# Autodesk Inventor assembly: New Box ARm
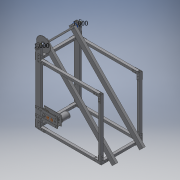
[picture p0: Inventor's stored thumbnail of the model, 180x180]
Saved by Autodesk Inventor 2018 (Build 220112000, 112)
## iProperties
Created: 2019-01-24
Part Number: New Box ARm
Document SubType Name: Assembly
Designer: Gabriel
Author: Gabriel
## Documents named in this file (18)
- C:\Users\Gabriel\Documents\GitHub\2019CAD\New ARm Box\New Box ARm.iam
- C:\Users\Gabriel\Documents\GitHub\2019CAD\New ARm Box\30in Vertical 1x2 Beam.ipt
- C:\Users\Gabriel\Documents\GitHub\2019CAD\New ARm Box\24in Vertical 1x1 Beam.ipt
- C:\Users\Gabriel\Documents\GitHub\2019CAD\New ARm Box\15in Horizontal 1x1 Beam.ipt
- C:\Users\Gabriel\Documents\GitHub\2019CAD\New ARm Box\24in Horizontal 1x1 Beam.ipt
- C:\Users\Gabriel\Documents\GitHub\2019CAD\New ARm Box\25in Horizontal 1x1 Beam.ipt
- C:\Users\Gabriel\Documents\GitHub\2019CAD\New ARm Box\ARm Gearbox.iam
- C:\Users\Gabriel\Documents\GitHub\2019CAD\New ARm Box\L gusset.ipt
- C:\Users\Gabriel\Documents\GitHub\2019CAD\New ARm Box\1_2_Acetal_Spacer_-_1_2_Hex_217-3261.ipt
- C:\Users\Gabriel\Documents\GitHub\2019CAD\New ARm Box\Clamping_Shaft_Collar_-_1_2_Hex_ID_217-2737.ipt
- C:\Users\Gabriel\Documents\GitHub\2019CAD\New ARm Box\_72t_Aluminum_Plate_Sprocket_25_Chain_1-1_8_Bearing_Bore_217-2627.ipt
- C:\Users\Gabriel\Documents\GitHub\2019CAD\New ARm Box\0_500_ID_x_1_125_OD_x_0_313_WD_Flanged_Bearing_217-2731.ipt
- C:\Users\Gabriel\Documents\GitHub\2019CAD\New ARm Box\41.75in Arm Beam.ipt
- C:\Users\Gabriel\Documents\GitHub\2019CAD\New ARm Box\Hex Hub.ipt
- C:\Users\Gabriel\Documents\GitHub\2019CAD\New ARm Box\Hex Shaft ARm.ipt
- C:\Users\Gabriel\Documents\GitHub\2019CAD\New ARm Box\.75in 92196A245_18-8 STAINLESS STEEL SOCKET HEAD CAP SCREW.ipt
- C:\Users\Gabriel\Documents\GitHub\2019CAD\New ARm Box\1.5in 92196A251_18-8 STAINLESS STEEL SOCKET HEAD CAP SCREW.ipt
- C:\Users\Gabriel\Downloads\LV Gusset.ipt
## Components (105 placed, 17 different names)
1. 30in Vertical 1x2 Beam:1 — Mate:4, Mate:5, Mate:6, Flush:6, Flush:17, Mate:27, Mate:30, Flush:19, Flush:21, Flush:31, Mate:38, Mate:39, Flush:35, Mate:41, Flush:43, Flush:44, Mate:53, Mate:54, Mate:55, Mate:56, Mate:57, Flush:60, Mate:58, Mate:60, Mate:61, Mate:62, Flush:61, Mate:65, Mate:67, Mate:68, Mate:69, Flush:64, Mate:79, Mate:81, Mate:82, Mate:83, Flush:68, Mate:93, Mate:95, Mate:96, Mate:97, Flush:72, Mate:168, Mate:177, Mate:178, Mate:179, Flush:110, Flush:114, Flush:118, Mate:184, Mate:186, Mate:187, Mate:188, Flush:122, Flush:125, Mate:196, Mate:197, Mate:198, Mate:199
2. 30in Vertical 1x2 Beam:2 — Mate:7, Mate:8, Mate:9, Flush:5, Flush:18, Mate:33, Mate:35, Flush:25, Flush:27, Flush:31, Mate:37, Mate:40, Flush:34, Mate:47, Flush:49, Flush:50, Mate:72, Mate:74, Mate:75, Mate:76, Flush:66, Mate:86, Mate:88, Mate:89, Mate:90, Flush:70, Mate:100, Mate:102, Mate:103, Mate:104, Flush:74, Mate:107, Mate:109, Mate:110, Mate:111, Flush:76, Mate:170, Mate:172, Mate:173, Mate:174, Flush:112, Flush:116, Flush:117, Mate:182, Mate:191, Mate:192, Mate:193, Flush:120, Flush:126, Mate:200, Mate:201, Mate:202, Mate:203
3. 24in Vertical 1x1 Beam:3 — Flush:13, Flush:16, Flush:17, Mate:28, Mate:29, Flush:20, Flush:22, Flush:23, Mate:31, Flush:39, Mate:45, Mate:46, Flush:40, Mate:114, Flush:78, Flush:79, Mate:128, Flush:84, Flush:85, Mate:156, Mate:158, Mate:159, Flush:100, Flush:103, Mate:300, Mate:304, Mate:305, Flush:134, Flush:135
4. 24in Vertical 1x1 Beam:4 — Flush:16, Flush:18, Mate:32, Mate:34, Flush:24, Flush:26, Flush:32, Mate:36, Mate:51, Mate:52, Flush:46, Flush:47, Mate:121, Flush:81, Flush:82, Mate:135, Flush:87, Flush:88, Mate:162, Mate:164, Mate:165, Flush:105, Flush:108, Mate:306, Mate:310, Mate:311, Flush:130, Flush:131
5. 15in Horizontal 1x1 Beam:1 — Flush:13, Flush:30, Mate:42, Mate:43, Mate:44, Flush:41, Flush:42, Mate:48, Flush:45, Mate:49, Mate:50, Flush:48, Flush:52, Flush:53, Flush:56, Mate:157, Mate:160, Mate:161, Flush:99, Flush:101, Mate:163, Mate:166, Mate:167, Flush:104, Flush:106, Mate:242
6. 15in Horizontal 1x1 Beam:2 — Mate:4, Mate:5, Mate:6, Mate:7, Mate:8, Mate:9, Flush:5, Flush:6, Flush:30, Flush:38, Flush:54, Flush:55, Flush:56, Mate:169, Mate:171, Mate:175, Mate:176, Mate:180, Mate:181, Flush:109, Flush:111, Flush:113, Flush:115
7. 15in Horizontal 1x1 Beam:3 — Mate:37, Mate:38, Mate:39, Mate:40, Flush:34, Flush:35, Flush:36, Flush:37, Flush:38, Mate:183, Mate:185, Mate:189, Mate:190, Mate:194, Mate:195, Flush:119, Flush:121, Flush:123, Flush:124
8. 24in Horizontal 1x1 Beam:1 — Mate:32, Mate:33, Mate:34, Mate:35, Flush:24, Flush:25, Flush:26, Flush:27, Flush:32, Mate:36, Flush:33, Flush:37, Flush:58, Mate:73, Mate:77, Mate:78, Flush:65, Mate:87, Mate:91, Mate:92, Flush:69, Mate:122, Mate:123, Mate:124, Flush:80, Mate:136, Mate:137, Mate:138, Flush:86
9. 24in Horizontal 1x1 Beam:2 — Mate:27, Mate:28, Mate:29, Mate:30, Flush:19, Flush:20, Flush:21, Flush:22, Flush:23, Mate:31, Flush:33, Flush:36, Flush:57, Mate:66, Mate:70, Mate:71, Flush:63, Mate:80, Mate:84, Mate:85, Flush:67, Mate:115, Mate:116, Mate:117, Flush:77, Mate:129, Mate:130, Mate:131, Flush:83
10. 25in Horizontal 1x1 Beam:1 — Mate:41, Flush:39, Mate:42, Mate:43, Mate:44, Mate:45, Mate:46, Flush:40, Flush:41, Flush:42, Flush:43, Flush:44, Flush:51, Flush:53, Flush:55, Flush:57, Flush:59, Mate:59, Flush:62, Mate:94, Flush:71, Flush:102, Mate:301, Mate:302, Mate:303, Flush:133, Flush:136
11. 25in Horizontal 1x1 Beam:2 — Mate:47, Mate:48, Flush:45, Mate:49, Mate:50, Mate:51, Mate:52, Flush:46, Flush:47, Flush:48, Flush:49, Flush:50, Flush:51, Flush:52, Flush:54, Flush:58, Flush:59, Mate:101, Flush:73, Mate:108, Flush:75, Flush:107, Mate:307, Mate:308, Mate:309, Flush:129, Flush:132
12. ARm Gearbox:1 [sub-assembly] — Mate:53, Mate:54, Mate:55, Mate:56, Mate:57, Flush:60
13. L gusset:1 — Mate:93, Mate:94, Mate:95, Mate:96, Mate:97, Flush:71, Flush:72
14. L gusset:2 — Mate:100, Mate:101, Mate:102, Mate:103, Mate:104, Flush:73, Flush:74
15. L gusset:5 — Mate:114, Mate:115, Mate:116, Mate:117, Flush:77, Flush:78, Flush:79
16. L gusset:6 — Mate:121, Mate:122, Mate:123, Mate:124, Flush:80, Flush:81, Flush:82
17. L gusset:7 — Mate:72, Mate:73, Mate:74, Mate:75, Mate:76, Mate:77, Mate:78, Flush:65, Flush:66
18. L gusset:8 — Mate:65, Mate:66, Mate:67, Mate:68, Mate:69, Mate:70, Mate:71, Flush:63, Flush:64, Mate:273, Mate:274, Mate:275, Mate:277, Mate:289, Mate:291, Mate:292, Mate:293, Mate:382, Mate:383
19. L gusset:9 — Mate:58, Mate:59, Mate:60, Mate:61, Mate:62, Flush:61, Flush:62, Mate:259, Mate:260, Mate:261, Mate:263, Mate:285, Mate:286, Mate:287, Mate:288
20. L gusset:10 — Mate:107, Mate:108, Mate:109, Mate:110, Mate:111, Flush:75, Flush:76, Mate:296, Mate:297, Mate:298, Mate:328, Mate:329, Mate:330, Mate:337, Mate:338
21. L gusset:11 — Mate:86, Mate:87, Mate:88, Mate:89, Mate:90, Mate:91, Mate:92, Flush:69, Flush:70, Mate:364, Mate:365, Mate:366, Mate:368, Mate:369, Mate:370, Mate:372, Mate:373, Mate:380, Mate:381
22. L gusset:12 — Mate:79, Mate:80, Mate:81, Mate:82, Mate:83, Mate:84, Mate:85, Flush:67, Flush:68
23. L gusset:13 — Mate:135, Mate:136, Mate:137, Mate:138, Flush:86, Flush:87, Flush:88, Mate:332, Mate:333, Mate:334, Mate:335, Mate:336, Mate:359, Mate:360, Mate:361, Mate:362, Mate:363
24. L gusset:14 — Mate:128, Mate:129, Mate:130, Mate:131, Flush:83, Flush:84, Flush:85, Mate:268, Mate:269, Mate:270, Mate:271, Mate:272, Mate:278, Mate:279, Mate:280, Mate:281, Mate:282
25. L gusset:15 — Mate:168, Mate:169, Mate:177, Mate:178, Mate:179, Mate:180, Mate:181, Flush:109, Flush:110, Flush:113, Flush:114, Flush:118, Mate:339, Mate:340, Mate:341, Mate:342, Mate:349, Mate:350
26. L gusset:16 — Mate:156, Mate:157, Mate:158, Mate:159, Mate:160, Mate:161, Flush:99, Flush:100, Flush:101, Flush:102, Flush:103, Mate:351, Mate:352, Mate:357, Mate:358
27. L gusset:17 — Mate:184, Mate:185, Mate:186, Mate:187, Mate:188, Mate:189, Mate:190, Flush:121, Flush:122, Flush:123, Flush:125, Mate:376, Mate:377, Mate:388, Mate:389, Mate:390, Mate:391, Mate:394, Mate:395, Mate:400, Mate:401
28. L gusset:18 — Mate:162, Mate:163, Mate:164, Mate:165, Mate:166, Mate:167, Flush:104, Flush:105, Flush:106, Flush:107, Flush:108, Mate:353, Mate:354, Mate:355, Mate:356
29. L gusset:19 — Mate:170, Mate:171, Mate:172, Mate:173, Mate:174, Mate:175, Mate:176, Flush:111, Flush:112, Flush:115, Flush:116, Flush:117, Mate:343, Mate:344, Mate:345, Mate:346, Mate:347, Mate:348
30. L gusset:20 — Mate:182, Mate:183, Mate:191, Mate:192, Mate:193, Mate:194, Mate:195, Flush:119, Flush:120, Flush:124, Flush:126, Mate:384, Mate:385, Mate:386, Mate:387, Mate:392, Mate:393, Mate:396, Mate:397, Mate:398, Mate:399
31. 1_2_Acetal_Spacer_-_1_2_Hex_217-3261:1 — Mate:213, Mate:214, Mate:215, Mate:216
32. Clamping_Shaft_Collar_-_1_2_Hex_ID_217-2737:1 — Mate:204, Mate:205, Flush:127, Mate:208
33. _72t_Aluminum_Plate_Sprocket_25_Chain_1-1_8_Bearing_Bore_217-2627:1 — Mate:217, Mate:218, Mate:219, Mate:220, Mate:221
34. 0_500_ID_x_1_125_OD_x_0_313_WD_Flanged_Bearing_217-2731:1 — Mate:196, Mate:197, Mate:209, Mate:210
35. 1_2_Acetal_Spacer_-_1_2_Hex_217-3261:2 — Mate:206, Mate:207, Mate:208, Mate:209, Mate:210
36. 41.75in Arm Beam:1 — Mate:222, Mate:229, Flush:128, Rotation:3, Mate:242
37. 0_500_ID_x_1_125_OD_x_0_313_WD_Flanged_Bearing_217-2731:2 — Mate:198, Mate:199, Mate:215
38. Hex Hub:1 — Mate:211, Mate:212, Mate:216, Mate:217, Mate:218, Mate:219, Mate:220, Mate:221, Mate:226
39. Hex Hub:2 — Mate:222, Mate:224, Mate:225, Mate:226, Mate:229, Rotation:3, Rotation:4
40. Hex Shaft ARm:1 — Mate:204, Mate:205, Flush:127, Mate:206, Mate:207, Mate:211, Mate:212, Mate:213, Mate:214, Mate:224, Mate:225, Mate:230, Mate:231, Mate:233, Mate:234, Mate:236, Mate:237, Mate:240, Mate:241, Rotation:2, Rotation:4
41. 41.75in Arm Beam:2 — Mate:227, Mate:228, Rotation:1, Flush:128
42. Hex Hub:3 — Mate:227, Mate:228, Mate:239, Mate:240, Mate:241, Rotation:1, Rotation:2
43. 1_2_Acetal_Spacer_-_1_2_Hex_217-3261:4 — Mate:230, Mate:231, Mate:232, Mate:239
44. 0_500_ID_x_1_125_OD_x_0_313_WD_Flanged_Bearing_217-2731:3 — Mate:201, Mate:203, Mate:232
45. 0_500_ID_x_1_125_OD_x_0_313_WD_Flanged_Bearing_217-2731:4 — Mate:200, Mate:202, Mate:235
46. 1_2_Acetal_Spacer_-_1_2_Hex_217-3261:6 — Mate:233, Mate:234, Mate:235, Mate:238
47. Clamping_Shaft_Collar_-_1_2_Hex_ID_217-2737:2 — Mate:236, Mate:237, Mate:238
48. .75in 92196A245_18-8 STAINLESS STEEL SOCKET HEAD CAP SCREW:1 — Mate:376, Mate:377
49. 1.5in 92196A251_18-8 STAINLESS STEEL SOCKET HEAD CAP SCREW:1 — Mate:320, Mate:322
50. 1.5in 92196A251_18-8 STAINLESS STEEL SOCKET HEAD CAP SCREW:2 — Mate:317, Mate:319
51. 1.5in 92196A251_18-8 STAINLESS STEEL SOCKET HEAD CAP SCREW:3 — Mate:324, Mate:327
52. 1.5in 92196A251_18-8 STAINLESS STEEL SOCKET HEAD CAP SCREW:5 — Mate:341, Mate:350
53. 1.5in 92196A251_18-8 STAINLESS STEEL SOCKET HEAD CAP SCREW:6 — Mate:364, Mate:369
54. 1.5in 92196A251_18-8 STAINLESS STEEL SOCKET HEAD CAP SCREW:7 — Mate:312, Mate:315
55. 1.5in 92196A251_18-8 STAINLESS STEEL SOCKET HEAD CAP SCREW:8 — Mate:325, Mate:326
56. 1.5in 92196A251_18-8 STAINLESS STEEL SOCKET HEAD CAP SCREW:9 — Mate:271, Mate:281
57. 1.5in 92196A251_18-8 STAINLESS STEEL SOCKET HEAD CAP SCREW:10 — Mate:270, Mate:280
58. 1.5in 92196A251_18-8 STAINLESS STEEL SOCKET HEAD CAP SCREW:11 — Mate:313, Mate:314
59. 1.5in 92196A251_18-8 STAINLESS STEEL SOCKET HEAD CAP SCREW:12 — Mate:332, Mate:361
60. 1.5in 92196A251_18-8 STAINLESS STEEL SOCKET HEAD CAP SCREW:13 — Mate:259, Mate:288
61. .75in 92196A245_18-8 STAINLESS STEEL SOCKET HEAD CAP SCREW:14 — Mate:386, Mate:392
62. 1.5in 92196A251_18-8 STAINLESS STEEL SOCKET HEAD CAP SCREW:14 — Mate:316, Mate:318
63. .75in 92196A245_18-8 STAINLESS STEEL SOCKET HEAD CAP SCREW:15 — Mate:387, Mate:393
64. 1.5in 92196A251_18-8 STAINLESS STEEL SOCKET HEAD CAP SCREW:15 — Mate:297, Mate:329
65. .75in 92196A245_18-8 STAINLESS STEEL SOCKET HEAD CAP SCREW:17 — Mate:388, Mate:390
66. 1.5in 92196A251_18-8 STAINLESS STEEL SOCKET HEAD CAP SCREW:17 — Mate:298, Mate:330
67. 1.5in 92196A251_18-8 STAINLESS STEEL SOCKET HEAD CAP SCREW:18 — Mate:336, Mate:363
68. 1.5in 92196A251_18-8 STAINLESS STEEL SOCKET HEAD CAP SCREW:19 — Mate:366, Mate:372
69. 1.5in 92196A251_18-8 STAINLESS STEEL SOCKET HEAD CAP SCREW:20 — Mate:321, Mate:323
70. 1.5in 92196A251_18-8 STAINLESS STEEL SOCKET HEAD CAP SCREW:21 — Mate:339, Mate:340
71. 1.5in 92196A251_18-8 STAINLESS STEEL SOCKET HEAD CAP SCREW:22 — Mate:334, Mate:359
72. 1.5in 92196A251_18-8 STAINLESS STEEL SOCKET HEAD CAP SCREW:24 — Mate:261, Mate:286
73. 1.5in 92196A251_18-8 STAINLESS STEEL SOCKET HEAD CAP SCREW:25 — Mate:275, Mate:291
74. 1.5in 92196A251_18-8 STAINLESS STEEL SOCKET HEAD CAP SCREW:26 — Mate:333, Mate:360
75. 1.5in 92196A251_18-8 STAINLESS STEEL SOCKET HEAD CAP SCREW:27 — Mate:365, Mate:370
76. 1.5in 92196A251_18-8 STAINLESS STEEL SOCKET HEAD CAP SCREW:28 — Mate:337, Mate:338
77. 1.5in 92196A251_18-8 STAINLESS STEEL SOCKET HEAD CAP SCREW:30 — Mate:335, Mate:362
78. 1.5in 92196A251_18-8 STAINLESS STEEL SOCKET HEAD CAP SCREW:31 — Mate:368, Mate:373
79. 1.5in 92196A251_18-8 STAINLESS STEEL SOCKET HEAD CAP SCREW:33 — Mate:395, Mate:401
80. .75in 92196A245_18-8 STAINLESS STEEL SOCKET HEAD CAP SCREW:34 — Mate:384, Mate:385
81. 1.5in 92196A251_18-8 STAINLESS STEEL SOCKET HEAD CAP SCREW:34 — Mate:296, Mate:328
82. 1.5in 92196A251_18-8 STAINLESS STEEL SOCKET HEAD CAP SCREW:35 — Mate:273, Mate:293
83. 1.5in 92196A251_18-8 STAINLESS STEEL SOCKET HEAD CAP SCREW:36 — Mate:274, Mate:292
84. 1.5in 92196A251_18-8 STAINLESS STEEL SOCKET HEAD CAP SCREW:38 — Mate:263, Mate:287
85. 1.5in 92196A251_18-8 STAINLESS STEEL SOCKET HEAD CAP SCREW:39 — Mate:260, Mate:285
86. 1.5in 92196A251_18-8 STAINLESS STEEL SOCKET HEAD CAP SCREW:43 — Mate:277, Mate:289
87. 1.5in 92196A251_18-8 STAINLESS STEEL SOCKET HEAD CAP SCREW:45 — Mate:272, Mate:282
88. 1.5in 92196A251_18-8 STAINLESS STEEL SOCKET HEAD CAP SCREW:47 — Mate:269, Mate:278
89. 1.5in 92196A251_18-8 STAINLESS STEEL SOCKET HEAD CAP SCREW:49 — Mate:268, Mate:279
90. 1.5in 92196A251_18-8 STAINLESS STEEL SOCKET HEAD CAP SCREW:50 — Mate:397, Mate:399
91. 1.5in 92196A251_18-8 STAINLESS STEEL SOCKET HEAD CAP SCREW:51 — Mate:343, Mate:348
92. 1.5in 92196A251_18-8 STAINLESS STEEL SOCKET HEAD CAP SCREW:52 — Mate:342, Mate:349
93. 1.5in 92196A251_18-8 STAINLESS STEEL SOCKET HEAD CAP SCREW:54 — Mate:394, Mate:400
94. 1.5in 92196A251_18-8 STAINLESS STEEL SOCKET HEAD CAP SCREW:56 — Mate:396, Mate:398
95. LV Gusset:1 — Mate:306, Mate:307, Mate:308, Mate:309, Mate:310, Mate:311, Flush:129, Flush:130, Flush:131, Flush:132, Mate:320, Mate:321, Mate:322, Mate:323, Mate:324, Mate:325, Mate:326, Mate:327
96. LV Gusset:2 — Mate:300, Mate:301, Mate:302, Mate:303, Mate:304, Mate:305, Flush:133, Flush:134, Flush:135, Flush:136, Mate:312, Mate:313, Mate:314, Mate:315, Mate:316, Mate:317, Mate:318, Mate:319
97. 1.5in 92196A251_18-8 STAINLESS STEEL SOCKET HEAD CAP SCREW:58 — Mate:344, Mate:347
98. 1.5in 92196A251_18-8 STAINLESS STEEL SOCKET HEAD CAP SCREW:59 — Mate:345, Mate:346
99. 1.5in 92196A251_18-8 STAINLESS STEEL SOCKET HEAD CAP SCREW:60 — Mate:354, Mate:355
100. 1.5in 92196A251_18-8 STAINLESS STEEL SOCKET HEAD CAP SCREW:61 — Mate:352, Mate:358
101. 1.5in 92196A251_18-8 STAINLESS STEEL SOCKET HEAD CAP SCREW:64 — Mate:353, Mate:356
102. 1.5in 92196A251_18-8 STAINLESS STEEL SOCKET HEAD CAP SCREW:67 — Mate:351, Mate:357
103. 1.5in 92196A251_18-8 STAINLESS STEEL SOCKET HEAD CAP SCREW:68 — Mate:380, Mate:381
104. 1.5in 92196A251_18-8 STAINLESS STEEL SOCKET HEAD CAP SCREW:69 — Mate:382, Mate:383
105. .75in 92196A245_18-8 STAINLESS STEEL SOCKET HEAD CAP SCREW:58 — Mate:389, Mate:391
## Relationships (427: Mate 311, Flush 112, RelateRotation 4)
- Mate:4: 30in Vertical 1x2 Beam:1 ↔ 15in Horizontal 1x1 Beam:2
- Mate:5: 30in Vertical 1x2 Beam:1 ↔ 15in Horizontal 1x1 Beam:2
- Mate:6: 30in Vertical 1x2 Beam:1 ↔ 15in Horizontal 1x1 Beam:2
- Mate:7: 30in Vertical 1x2 Beam:2 ↔ 15in Horizontal 1x1 Beam:2
- Mate:8: 30in Vertical 1x2 Beam:2 ↔ 15in Horizontal 1x1 Beam:2
- Mate:9: 30in Vertical 1x2 Beam:2 ↔ 15in Horizontal 1x1 Beam:2
- Flush:5: 30in Vertical 1x2 Beam:2 ↔ 15in Horizontal 1x1 Beam:2
- Flush:6: 30in Vertical 1x2 Beam:1 ↔ 15in Horizontal 1x1 Beam:2
- Flush:13: 24in Vertical 1x1 Beam:3 ↔ 15in Horizontal 1x1 Beam:1
- Flush:16: 24in Vertical 1x1 Beam:3 ↔ 24in Vertical 1x1 Beam:4
- Flush:17: 30in Vertical 1x2 Beam:1 ↔ 24in Vertical 1x1 Beam:3
- Flush:18: 30in Vertical 1x2 Beam:2 ↔ 24in Vertical 1x1 Beam:4
- Mate:27: 30in Vertical 1x2 Beam:1 ↔ 24in Horizontal 1x1 Beam:2
- Mate:28: 24in Vertical 1x1 Beam:3 ↔ 24in Horizontal 1x1 Beam:2
- Mate:29: 24in Vertical 1x1 Beam:3 ↔ 24in Horizontal 1x1 Beam:2
- Mate:30: 30in Vertical 1x2 Beam:1 ↔ 24in Horizontal 1x1 Beam:2
- Flush:19: 30in Vertical 1x2 Beam:1 ↔ 24in Horizontal 1x1 Beam:2
- Flush:20: 24in Vertical 1x1 Beam:3 ↔ 24in Horizontal 1x1 Beam:2
- Flush:21: 30in Vertical 1x2 Beam:1 ↔ 24in Horizontal 1x1 Beam:2
- Flush:22: 24in Vertical 1x1 Beam:3 ↔ 24in Horizontal 1x1 Beam:2
- Flush:23: 24in Vertical 1x1 Beam:3 ↔ 24in Horizontal 1x1 Beam:2
- Mate:31: 24in Vertical 1x1 Beam:3 ↔ 24in Horizontal 1x1 Beam:2
- Mate:32: 24in Vertical 1x1 Beam:4 ↔ 24in Horizontal 1x1 Beam:1
- Mate:33: 30in Vertical 1x2 Beam:2 ↔ 24in Horizontal 1x1 Beam:1
- Mate:34: 24in Vertical 1x1 Beam:4 ↔ 24in Horizontal 1x1 Beam:1
- Mate:35: 30in Vertical 1x2 Beam:2 ↔ 24in Horizontal 1x1 Beam:1
- Flush:24: 24in Vertical 1x1 Beam:4 ↔ 24in Horizontal 1x1 Beam:1
- Flush:25: 30in Vertical 1x2 Beam:2 ↔ 24in Horizontal 1x1 Beam:1
- Flush:26: 24in Vertical 1x1 Beam:4 ↔ 24in Horizontal 1x1 Beam:1
- Flush:27: 30in Vertical 1x2 Beam:2 ↔ 24in Horizontal 1x1 Beam:1
- Flush:30: 15in Horizontal 1x1 Beam:1 ↔ 15in Horizontal 1x1 Beam:2
- Flush:31: 30in Vertical 1x2 Beam:1 ↔ 30in Vertical 1x2 Beam:2
- Flush:32: 24in Vertical 1x1 Beam:4 ↔ 24in Horizontal 1x1 Beam:1
- Mate:36: 24in Vertical 1x1 Beam:4 ↔ 24in Horizontal 1x1 Beam:1
- Flush:33: 24in Horizontal 1x1 Beam:1 ↔ 24in Horizontal 1x1 Beam:2
- Mate:37: 30in Vertical 1x2 Beam:2 ↔ 15in Horizontal 1x1 Beam:3
- Mate:38: 30in Vertical 1x2 Beam:1 ↔ 15in Horizontal 1x1 Beam:3
- Mate:39: 30in Vertical 1x2 Beam:1 ↔ 15in Horizontal 1x1 Beam:3
- Mate:40: 30in Vertical 1x2 Beam:2 ↔ 15in Horizontal 1x1 Beam:3
- Flush:34: 30in Vertical 1x2 Beam:2 ↔ 15in Horizontal 1x1 Beam:3
- Flush:35: 30in Vertical 1x2 Beam:1 ↔ 15in Horizontal 1x1 Beam:3
- Flush:36: 15in Horizontal 1x1 Beam:3 ↔ 24in Horizontal 1x1 Beam:2
- Flush:37: 15in Horizontal 1x1 Beam:3 ↔ 24in Horizontal 1x1 Beam:1
- Flush:38: 15in Horizontal 1x1 Beam:2 ↔ 15in Horizontal 1x1 Beam:3
- Mate:41: 30in Vertical 1x2 Beam:1 ↔ 25in Horizontal 1x1 Beam:1
- Flush:39: 24in Vertical 1x1 Beam:3 ↔ 25in Horizontal 1x1 Beam:1
- Mate:42: 15in Horizontal 1x1 Beam:1 ↔ 25in Horizontal 1x1 Beam:1
- Mate:43: 15in Horizontal 1x1 Beam:1 ↔ 25in Horizontal 1x1 Beam:1
- Mate:44: 15in Horizontal 1x1 Beam:1 ↔ 25in Horizontal 1x1 Beam:1
- Mate:45: 24in Vertical 1x1 Beam:3 ↔ 25in Horizontal 1x1 Beam:1
- Mate:46: 24in Vertical 1x1 Beam:3 ↔ 25in Horizontal 1x1 Beam:1
- Flush:40: 24in Vertical 1x1 Beam:3 ↔ 25in Horizontal 1x1 Beam:1
- Flush:41: 15in Horizontal 1x1 Beam:1 ↔ 25in Horizontal 1x1 Beam:1
- Flush:42: 15in Horizontal 1x1 Beam:1 ↔ 25in Horizontal 1x1 Beam:1
- Flush:43: 30in Vertical 1x2 Beam:1 ↔ 25in Horizontal 1x1 Beam:1
- Flush:44: 30in Vertical 1x2 Beam:1 ↔ 25in Horizontal 1x1 Beam:1
- Mate:47: 30in Vertical 1x2 Beam:2 ↔ 25in Horizontal 1x1 Beam:2
- Mate:48: 15in Horizontal 1x1 Beam:1 ↔ 25in Horizontal 1x1 Beam:2
- Flush:45: 15in Horizontal 1x1 Beam:1 ↔ 25in Horizontal 1x1 Beam:2
- Mate:49: 15in Horizontal 1x1 Beam:1 ↔ 25in Horizontal 1x1 Beam:2
- Mate:50: 15in Horizontal 1x1 Beam:1 ↔ 25in Horizontal 1x1 Beam:2
- Mate:51: 24in Vertical 1x1 Beam:4 ↔ 25in Horizontal 1x1 Beam:2
- Mate:52: 24in Vertical 1x1 Beam:4 ↔ 25in Horizontal 1x1 Beam:2
- Flush:46: 24in Vertical 1x1 Beam:4 ↔ 25in Horizontal 1x1 Beam:2
- Flush:47: 24in Vertical 1x1 Beam:4 ↔ 25in Horizontal 1x1 Beam:2
- Flush:48: 15in Horizontal 1x1 Beam:1 ↔ 25in Horizontal 1x1 Beam:2
- Flush:49: 30in Vertical 1x2 Beam:2 ↔ 25in Horizontal 1x1 Beam:2
- Flush:50: 30in Vertical 1x2 Beam:2 ↔ 25in Horizontal 1x1 Beam:2
- Flush:51: 25in Horizontal 1x1 Beam:1 ↔ 25in Horizontal 1x1 Beam:2
- Flush:52: 15in Horizontal 1x1 Beam:1 ↔ 25in Horizontal 1x1 Beam:2
- Flush:53: 15in Horizontal 1x1 Beam:1 ↔ 25in Horizontal 1x1 Beam:1
- Flush:54: 15in Horizontal 1x1 Beam:2 ↔ 25in Horizontal 1x1 Beam:2
- Flush:55: 15in Horizontal 1x1 Beam:2 ↔ 25in Horizontal 1x1 Beam:1
- Flush:56: 15in Horizontal 1x1 Beam:1 ↔ 15in Horizontal 1x1 Beam:2
- Flush:57: 24in Horizontal 1x1 Beam:2 ↔ 25in Horizontal 1x1 Beam:1
- Flush:58: 24in Horizontal 1x1 Beam:1 ↔ 25in Horizontal 1x1 Beam:2
- Flush:59: 25in Horizontal 1x1 Beam:1 ↔ 25in Horizontal 1x1 Beam:2
- Mate:53: 30in Vertical 1x2 Beam:1 ↔ ARm Gearbox:1
- Mate:54: 30in Vertical 1x2 Beam:1 ↔ ARm Gearbox:1
- Mate:55: 30in Vertical 1x2 Beam:1 ↔ ARm Gearbox:1
- Mate:56: 30in Vertical 1x2 Beam:1 ↔ ARm Gearbox:1
- Mate:57: 30in Vertical 1x2 Beam:1 ↔ ARm Gearbox:1
- Flush:60: 30in Vertical 1x2 Beam:1 ↔ ARm Gearbox:1
- Mate:58: 30in Vertical 1x2 Beam:1 ↔ L gusset:9
- Mate:59: 25in Horizontal 1x1 Beam:1 ↔ L gusset:9
- Mate:60: 30in Vertical 1x2 Beam:1 ↔ L gusset:9
- Mate:61: 30in Vertical 1x2 Beam:1 ↔ L gusset:9
- Mate:62: 30in Vertical 1x2 Beam:1 ↔ L gusset:9
- Flush:61: 30in Vertical 1x2 Beam:1 ↔ L gusset:9
- Flush:62: 25in Horizontal 1x1 Beam:1 ↔ L gusset:9
- Mate:65: 30in Vertical 1x2 Beam:1 ↔ L gusset:8
- Mate:66: 24in Horizontal 1x1 Beam:2 ↔ L gusset:8
- Mate:67: 30in Vertical 1x2 Beam:1 ↔ L gusset:8
- Mate:68: 30in Vertical 1x2 Beam:1 ↔ L gusset:8
- Mate:69: 30in Vertical 1x2 Beam:1 ↔ L gusset:8
- Mate:70: 24in Horizontal 1x1 Beam:2 ↔ L gusset:8
- Mate:71: 24in Horizontal 1x1 Beam:2 ↔ L gusset:8
- Flush:63: 24in Horizontal 1x1 Beam:2 ↔ L gusset:8
- Flush:64: 30in Vertical 1x2 Beam:1 ↔ L gusset:8
- Mate:72: 30in Vertical 1x2 Beam:2 ↔ L gusset:7
- Mate:73: 24in Horizontal 1x1 Beam:1 ↔ L gusset:7
- Mate:74: 30in Vertical 1x2 Beam:2 ↔ L gusset:7
- Mate:75: 30in Vertical 1x2 Beam:2 ↔ L gusset:7
- Mate:76: 30in Vertical 1x2 Beam:2 ↔ L gusset:7
- Mate:77: 24in Horizontal 1x1 Beam:1 ↔ L gusset:7
- Mate:78: 24in Horizontal 1x1 Beam:1 ↔ L gusset:7
- Flush:65: 24in Horizontal 1x1 Beam:1 ↔ L gusset:7
- Flush:66: 30in Vertical 1x2 Beam:2 ↔ L gusset:7
- Mate:79: 30in Vertical 1x2 Beam:1 ↔ L gusset:12
- Mate:80: 24in Horizontal 1x1 Beam:2 ↔ L gusset:12
- Mate:81: 30in Vertical 1x2 Beam:1 ↔ L gusset:12
- Mate:82: 30in Vertical 1x2 Beam:1 ↔ L gusset:12
- Mate:83: 30in Vertical 1x2 Beam:1 ↔ L gusset:12
- Mate:84: 24in Horizontal 1x1 Beam:2 ↔ L gusset:12
- Mate:85: 24in Horizontal 1x1 Beam:2 ↔ L gusset:12
- Flush:67: 24in Horizontal 1x1 Beam:2 ↔ L gusset:12
- Flush:68: 30in Vertical 1x2 Beam:1 ↔ L gusset:12
- Mate:86: 30in Vertical 1x2 Beam:2 ↔ L gusset:11
- Mate:87: 24in Horizontal 1x1 Beam:1 ↔ L gusset:11
- Mate:88: 30in Vertical 1x2 Beam:2 ↔ L gusset:11
- Mate:89: 30in Vertical 1x2 Beam:2 ↔ L gusset:11
- Mate:90: 30in Vertical 1x2 Beam:2 ↔ L gusset:11
- Mate:91: 24in Horizontal 1x1 Beam:1 ↔ L gusset:11
- Mate:92: 24in Horizontal 1x1 Beam:1 ↔ L gusset:11
- Flush:69: 24in Horizontal 1x1 Beam:1 ↔ L gusset:11
- Flush:70: 30in Vertical 1x2 Beam:2 ↔ L gusset:11
- Mate:93: 30in Vertical 1x2 Beam:1 ↔ L gusset:1
- Mate:94: 25in Horizontal 1x1 Beam:1 ↔ L gusset:1
- Mate:95: 30in Vertical 1x2 Beam:1 ↔ L gusset:1
- Mate:96: 30in Vertical 1x2 Beam:1 ↔ L gusset:1
- Mate:97: 30in Vertical 1x2 Beam:1 ↔ L gusset:1
- Flush:71: 25in Horizontal 1x1 Beam:1 ↔ L gusset:1
- Flush:72: 30in Vertical 1x2 Beam:1 ↔ L gusset:1
- Mate:100: 30in Vertical 1x2 Beam:2 ↔ L gusset:2
- Mate:101: 25in Horizontal 1x1 Beam:2 ↔ L gusset:2
- Mate:102: 30in Vertical 1x2 Beam:2 ↔ L gusset:2
- Mate:103: 30in Vertical 1x2 Beam:2 ↔ L gusset:2
- Mate:104: 30in Vertical 1x2 Beam:2 ↔ L gusset:2
- Flush:73: 25in Horizontal 1x1 Beam:2 ↔ L gusset:2
- Flush:74: 30in Vertical 1x2 Beam:2 ↔ L gusset:2
- Mate:107: 30in Vertical 1x2 Beam:2 ↔ L gusset:10
- Mate:108: 25in Horizontal 1x1 Beam:2 ↔ L gusset:10
- Mate:109: 30in Vertical 1x2 Beam:2 ↔ L gusset:10
- Mate:110: 30in Vertical 1x2 Beam:2 ↔ L gusset:10
- Mate:111: 30in Vertical 1x2 Beam:2 ↔ L gusset:10
- Flush:75: 25in Horizontal 1x1 Beam:2 ↔ L gusset:10
- Flush:76: 30in Vertical 1x2 Beam:2 ↔ L gusset:10
- Mate:114: 24in Vertical 1x1 Beam:3 ↔ L gusset:5
- Mate:115: 24in Horizontal 1x1 Beam:2 ↔ L gusset:5
- Mate:116: 24in Horizontal 1x1 Beam:2 ↔ L gusset:5
- Mate:117: 24in Horizontal 1x1 Beam:2 ↔ L gusset:5
- Flush:77: 24in Horizontal 1x1 Beam:2 ↔ L gusset:5
- Flush:78: 24in Vertical 1x1 Beam:3 ↔ L gusset:5
- Flush:79: 24in Vertical 1x1 Beam:3 ↔ L gusset:5
- Mate:121: 24in Vertical 1x1 Beam:4 ↔ L gusset:6
- Mate:122: 24in Horizontal 1x1 Beam:1 ↔ L gusset:6
- Mate:123: 24in Horizontal 1x1 Beam:1 ↔ L gusset:6
- Mate:124: 24in Horizontal 1x1 Beam:1 ↔ L gusset:6
- Flush:80: 24in Horizontal 1x1 Beam:1 ↔ L gusset:6
- Flush:81: 24in Vertical 1x1 Beam:4 ↔ L gusset:6
- Flush:82: 24in Vertical 1x1 Beam:4 ↔ L gusset:6
- Mate:128: 24in Vertical 1x1 Beam:3 ↔ L gusset:14
- Mate:129: 24in Horizontal 1x1 Beam:2 ↔ L gusset:14
- Mate:130: 24in Horizontal 1x1 Beam:2 ↔ L gusset:14
- Mate:131: 24in Horizontal 1x1 Beam:2 ↔ L gusset:14
- Flush:83: 24in Horizontal 1x1 Beam:2 ↔ L gusset:14
- Flush:84: 24in Vertical 1x1 Beam:3 ↔ L gusset:14
- Flush:85: 24in Vertical 1x1 Beam:3 ↔ L gusset:14
- Mate:135: 24in Vertical 1x1 Beam:4 ↔ L gusset:13
- Mate:136: 24in Horizontal 1x1 Beam:1 ↔ L gusset:13
- Mate:137: 24in Horizontal 1x1 Beam:1 ↔ L gusset:13
- Mate:138: 24in Horizontal 1x1 Beam:1 ↔ L gusset:13
- Flush:86: 24in Horizontal 1x1 Beam:1 ↔ L gusset:13
- Flush:87: 24in Vertical 1x1 Beam:4 ↔ L gusset:13
- Flush:88: 24in Vertical 1x1 Beam:4 ↔ L gusset:13
- Mate:156: 24in Vertical 1x1 Beam:3 ↔ L gusset:16
- Mate:157: 15in Horizontal 1x1 Beam:1 ↔ L gusset:16
- Mate:158: 24in Vertical 1x1 Beam:3 ↔ L gusset:16
- Mate:159: 24in Vertical 1x1 Beam:3 ↔ L gusset:16
- Mate:160: 15in Horizontal 1x1 Beam:1 ↔ L gusset:16
- Mate:161: 15in Horizontal 1x1 Beam:1 ↔ L gusset:16
- Flush:99: 15in Horizontal 1x1 Beam:1 ↔ L gusset:16
- Flush:100: 24in Vertical 1x1 Beam:3 ↔ L gusset:16
- Flush:101: 15in Horizontal 1x1 Beam:1 ↔ L gusset:16
- Flush:102: 25in Horizontal 1x1 Beam:1 ↔ L gusset:16
- Flush:103: 24in Vertical 1x1 Beam:3 ↔ L gusset:16
- Mate:162: 24in Vertical 1x1 Beam:4 ↔ L gusset:18
- Mate:163: 15in Horizontal 1x1 Beam:1 ↔ L gusset:18
- Mate:164: 24in Vertical 1x1 Beam:4 ↔ L gusset:18
- Mate:165: 24in Vertical 1x1 Beam:4 ↔ L gusset:18
- Mate:166: 15in Horizontal 1x1 Beam:1 ↔ L gusset:18
- Mate:167: 15in Horizontal 1x1 Beam:1 ↔ L gusset:18
- Flush:104: 15in Horizontal 1x1 Beam:1 ↔ L gusset:18
- Flush:105: 24in Vertical 1x1 Beam:4 ↔ L gusset:18
- Flush:106: 15in Horizontal 1x1 Beam:1 ↔ L gusset:18
- Flush:107: 25in Horizontal 1x1 Beam:2 ↔ L gusset:18
- Flush:108: 24in Vertical 1x1 Beam:4 ↔ L gusset:18
- Mate:168: 30in Vertical 1x2 Beam:1 ↔ L gusset:15
- Mate:169: 15in Horizontal 1x1 Beam:2 ↔ L gusset:15
- Mate:170: 30in Vertical 1x2 Beam:2 ↔ L gusset:19
- Mate:171: 15in Horizontal 1x1 Beam:2 ↔ L gusset:19
- Mate:172: 30in Vertical 1x2 Beam:2 ↔ L gusset:19
- Mate:173: 30in Vertical 1x2 Beam:2 ↔ L gusset:19
- Mate:174: 30in Vertical 1x2 Beam:2 ↔ L gusset:19
- Mate:175: 15in Horizontal 1x1 Beam:2 ↔ L gusset:19
- Mate:176: 15in Horizontal 1x1 Beam:2 ↔ L gusset:19
- Mate:177: 30in Vertical 1x2 Beam:1 ↔ L gusset:15
- Mate:178: 30in Vertical 1x2 Beam:1 ↔ L gusset:15
- Mate:179: 30in Vertical 1x2 Beam:1 ↔ L gusset:15
- Mate:180: 15in Horizontal 1x1 Beam:2 ↔ L gusset:15
- Mate:181: 15in Horizontal 1x1 Beam:2 ↔ L gusset:15
- Flush:109: 15in Horizontal 1x1 Beam:2 ↔ L gusset:15
- Flush:110: 30in Vertical 1x2 Beam:1 ↔ L gusset:15
- Flush:111: 15in Horizontal 1x1 Beam:2 ↔ L gusset:19
- Flush:112: 30in Vertical 1x2 Beam:2 ↔ L gusset:19
- Flush:113: 15in Horizontal 1x1 Beam:2 ↔ L gusset:15
- Flush:114: 30in Vertical 1x2 Beam:1 ↔ L gusset:15
- Flush:115: 15in Horizontal 1x1 Beam:2 ↔ L gusset:19
- Flush:116: 30in Vertical 1x2 Beam:2 ↔ L gusset:19
- Flush:117: 30in Vertical 1x2 Beam:2 ↔ L gusset:19
- Flush:118: 30in Vertical 1x2 Beam:1 ↔ L gusset:15
- Mate:182: 30in Vertical 1x2 Beam:2 ↔ L gusset:20
- Mate:183: 15in Horizontal 1x1 Beam:3 ↔ L gusset:20
- Mate:184: 30in Vertical 1x2 Beam:1 ↔ L gusset:17
- Mate:185: 15in Horizontal 1x1 Beam:3 ↔ L gusset:17
- Mate:186: 30in Vertical 1x2 Beam:1 ↔ L gusset:17
- Mate:187: 30in Vertical 1x2 Beam:1 ↔ L gusset:17
- Mate:188: 30in Vertical 1x2 Beam:1 ↔ L gusset:17
- Mate:189: 15in Horizontal 1x1 Beam:3 ↔ L gusset:17
- Mate:190: 15in Horizontal 1x1 Beam:3 ↔ L gusset:17
- Mate:191: 30in Vertical 1x2 Beam:2 ↔ L gusset:20
- Mate:192: 30in Vertical 1x2 Beam:2 ↔ L gusset:20
- Mate:193: 30in Vertical 1x2 Beam:2 ↔ L gusset:20
- Mate:194: 15in Horizontal 1x1 Beam:3 ↔ L gusset:20
- Mate:195: 15in Horizontal 1x1 Beam:3 ↔ L gusset:20
- Flush:119: 15in Horizontal 1x1 Beam:3 ↔ L gusset:20
- Flush:120: 30in Vertical 1x2 Beam:2 ↔ L gusset:20
- Flush:121: 15in Horizontal 1x1 Beam:3 ↔ L gusset:17
- Flush:122: 30in Vertical 1x2 Beam:1 ↔ L gusset:17
- Flush:123: 15in Horizontal 1x1 Beam:3 ↔ L gusset:17
- Flush:124: 15in Horizontal 1x1 Beam:3 ↔ L gusset:20
- Flush:125: 30in Vertical 1x2 Beam:1 ↔ L gusset:17
- Flush:126: 30in Vertical 1x2 Beam:2 ↔ L gusset:20
- Mate:196: 30in Vertical 1x2 Beam:1 ↔ 0_500_ID_x_1_125_OD_x_0_313_WD_Flanged_Bearing_217-2731:1
- Mate:197: 30in Vertical 1x2 Beam:1 ↔ 0_500_ID_x_1_125_OD_x_0_313_WD_Flanged_Bearing_217-2731:1
- Mate:198: 30in Vertical 1x2 Beam:1 ↔ 0_500_ID_x_1_125_OD_x_0_313_WD_Flanged_Bearing_217-2731:2
- Mate:199: 30in Vertical 1x2 Beam:1 ↔ 0_500_ID_x_1_125_OD_x_0_313_WD_Flanged_Bearing_217-2731:2
- Mate:200: 30in Vertical 1x2 Beam:2 ↔ 0_500_ID_x_1_125_OD_x_0_313_WD_Flanged_Bearing_217-2731:4
- Mate:201: 30in Vertical 1x2 Beam:2 ↔ 0_500_ID_x_1_125_OD_x_0_313_WD_Flanged_Bearing_217-2731:3
- Mate:202: 30in Vertical 1x2 Beam:2 ↔ 0_500_ID_x_1_125_OD_x_0_313_WD_Flanged_Bearing_217-2731:4
- Mate:203: 30in Vertical 1x2 Beam:2 ↔ 0_500_ID_x_1_125_OD_x_0_313_WD_Flanged_Bearing_217-2731:3
- Mate:204: Clamping_Shaft_Collar_-_1_2_Hex_ID_217-2737:1 ↔ Hex Shaft ARm:1
- Mate:205: Clamping_Shaft_Collar_-_1_2_Hex_ID_217-2737:1 ↔ Hex Shaft ARm:1
- Flush:127: Clamping_Shaft_Collar_-_1_2_Hex_ID_217-2737:1 ↔ Hex Shaft ARm:1
- Mate:206: 1_2_Acetal_Spacer_-_1_2_Hex_217-3261:2 ↔ Hex Shaft ARm:1
- Mate:207: 1_2_Acetal_Spacer_-_1_2_Hex_217-3261:2 ↔ Hex Shaft ARm:1
- Mate:208: Clamping_Shaft_Collar_-_1_2_Hex_ID_217-2737:1 ↔ 1_2_Acetal_Spacer_-_1_2_Hex_217-3261:2
- Mate:209: 0_500_ID_x_1_125_OD_x_0_313_WD_Flanged_Bearing_217-2731:1 ↔ 1_2_Acetal_Spacer_-_1_2_Hex_217-3261:2
- Mate:210: 0_500_ID_x_1_125_OD_x_0_313_WD_Flanged_Bearing_217-2731:1 ↔ 1_2_Acetal_Spacer_-_1_2_Hex_217-3261:2
- Mate:211: Hex Hub:1 ↔ Hex Shaft ARm:1
- Mate:212: Hex Hub:1 ↔ Hex Shaft ARm:1
- Mate:213: 1_2_Acetal_Spacer_-_1_2_Hex_217-3261:1 ↔ Hex Shaft ARm:1
- Mate:214: 1_2_Acetal_Spacer_-_1_2_Hex_217-3261:1 ↔ Hex Shaft ARm:1
- Mate:215: 1_2_Acetal_Spacer_-_1_2_Hex_217-3261:1 ↔ 0_500_ID_x_1_125_OD_x_0_313_WD_Flanged_Bearing_217-2731:2
- Mate:216: 1_2_Acetal_Spacer_-_1_2_Hex_217-3261:1 ↔ Hex Hub:1
- Mate:217: _72t_Aluminum_Plate_Sprocket_25_Chain_1-1_8_Bearing_Bore_217-2627:1 ↔ Hex Hub:1
- Mate:218: _72t_Aluminum_Plate_Sprocket_25_Chain_1-1_8_Bearing_Bore_217-2627:1 ↔ Hex Hub:1
- Mate:219: _72t_Aluminum_Plate_Sprocket_25_Chain_1-1_8_Bearing_Bore_217-2627:1 ↔ Hex Hub:1
- Mate:220: _72t_Aluminum_Plate_Sprocket_25_Chain_1-1_8_Bearing_Bore_217-2627:1 ↔ Hex Hub:1
- Mate:221: _72t_Aluminum_Plate_Sprocket_25_Chain_1-1_8_Bearing_Bore_217-2627:1 ↔ Hex Hub:1
- Mate:222: 41.75in Arm Beam:1 ↔ Hex Hub:2
- Mate:224: Hex Hub:2 ↔ Hex Shaft ARm:1
- Mate:225: Hex Hub:2 ↔ Hex Shaft ARm:1
- Mate:226: Hex Hub:1 ↔ Hex Hub:2
- Mate:227: 41.75in Arm Beam:2 ↔ Hex Hub:3
- Mate:228: 41.75in Arm Beam:2 ↔ Hex Hub:3
- Mate:229: 41.75in Arm Beam:1 ↔ Hex Hub:2
- Mate:230: Hex Shaft ARm:1 ↔ 1_2_Acetal_Spacer_-_1_2_Hex_217-3261:4
- Mate:231: Hex Shaft ARm:1 ↔ 1_2_Acetal_Spacer_-_1_2_Hex_217-3261:4
- Mate:232: 1_2_Acetal_Spacer_-_1_2_Hex_217-3261:4 ↔ 0_500_ID_x_1_125_OD_x_0_313_WD_Flanged_Bearing_217-2731:3
- Mate:233: Hex Shaft ARm:1 ↔ 1_2_Acetal_Spacer_-_1_2_Hex_217-3261:6
- Mate:234: Hex Shaft ARm:1 ↔ 1_2_Acetal_Spacer_-_1_2_Hex_217-3261:6
- Mate:235: 0_500_ID_x_1_125_OD_x_0_313_WD_Flanged_Bearing_217-2731:4 ↔ 1_2_Acetal_Spacer_-_1_2_Hex_217-3261:6
- Mate:236: Hex Shaft ARm:1 ↔ Clamping_Shaft_Collar_-_1_2_Hex_ID_217-2737:2
- Mate:237: Hex Shaft ARm:1 ↔ Clamping_Shaft_Collar_-_1_2_Hex_ID_217-2737:2
- Mate:238: 1_2_Acetal_Spacer_-_1_2_Hex_217-3261:6 ↔ Clamping_Shaft_Collar_-_1_2_Hex_ID_217-2737:2
- Mate:239: Hex Hub:3 ↔ 1_2_Acetal_Spacer_-_1_2_Hex_217-3261:4
- Mate:240: Hex Shaft ARm:1 ↔ Hex Hub:3
- Mate:241: Hex Shaft ARm:1 ↔ Hex Hub:3
- Rotation:1 [RelateRotation] (1 ul): 41.75in Arm Beam:2 ↔ Hex Hub:3
- Rotation:2 [RelateRotation] (1 ul): Hex Shaft ARm:1 ↔ Hex Hub:3
- Flush:128: 41.75in Arm Beam:1 ↔ 41.75in Arm Beam:2
- Rotation:3 [RelateRotation] (1 ul): 41.75in Arm Beam:1 ↔ Hex Hub:2
- Rotation:4 [RelateRotation] (1 ul): Hex Hub:2 ↔ Hex Shaft ARm:1
- Mate:242: 15in Horizontal 1x1 Beam:1 ↔ 41.75in Arm Beam:1
- Mate:259: L gusset:9 ↔ 1.5in 92196A251_18-8 STAINLESS STEEL SOCKET HEAD CAP SCREW:13
- Mate:260: L gusset:9 ↔ 1.5in 92196A251_18-8 STAINLESS STEEL SOCKET HEAD CAP SCREW:39
- Mate:261: L gusset:9 ↔ 1.5in 92196A251_18-8 STAINLESS STEEL SOCKET HEAD CAP SCREW:24
- Mate:263: L gusset:9 ↔ 1.5in 92196A251_18-8 STAINLESS STEEL SOCKET HEAD CAP SCREW:38
- Mate:268: L gusset:14 ↔ 1.5in 92196A251_18-8 STAINLESS STEEL SOCKET HEAD CAP SCREW:49
- Mate:269: L gusset:14 ↔ 1.5in 92196A251_18-8 STAINLESS STEEL SOCKET HEAD CAP SCREW:47
- Mate:270: L gusset:14 ↔ 1.5in 92196A251_18-8 STAINLESS STEEL SOCKET HEAD CAP SCREW:10
- Mate:271: L gusset:14 ↔ 1.5in 92196A251_18-8 STAINLESS STEEL SOCKET HEAD CAP SCREW:9
- Mate:272: L gusset:14 ↔ 1.5in 92196A251_18-8 STAINLESS STEEL SOCKET HEAD CAP SCREW:45
- Mate:273: L gusset:8 ↔ 1.5in 92196A251_18-8 STAINLESS STEEL SOCKET HEAD CAP SCREW:35
- Mate:274: L gusset:8 ↔ 1.5in 92196A251_18-8 STAINLESS STEEL SOCKET HEAD CAP SCREW:36
- Mate:275: L gusset:8 ↔ 1.5in 92196A251_18-8 STAINLESS STEEL SOCKET HEAD CAP SCREW:25
- Mate:277: L gusset:8 ↔ 1.5in 92196A251_18-8 STAINLESS STEEL SOCKET HEAD CAP SCREW:43
- Mate:278: L gusset:14 ↔ 1.5in 92196A251_18-8 STAINLESS STEEL SOCKET HEAD CAP SCREW:47
- Mate:279: L gusset:14 ↔ 1.5in 92196A251_18-8 STAINLESS STEEL SOCKET HEAD CAP SCREW:49
- Mate:280: L gusset:14 ↔ 1.5in 92196A251_18-8 STAINLESS STEEL SOCKET HEAD CAP SCREW:10
- Mate:281: L gusset:14 ↔ 1.5in 92196A251_18-8 STAINLESS STEEL SOCKET HEAD CAP SCREW:9
- Mate:282: L gusset:14 ↔ 1.5in 92196A251_18-8 STAINLESS STEEL SOCKET HEAD CAP SCREW:45
- Mate:285: L gusset:9 ↔ 1.5in 92196A251_18-8 STAINLESS STEEL SOCKET HEAD CAP SCREW:39
- Mate:286: L gusset:9 ↔ 1.5in 92196A251_18-8 STAINLESS STEEL SOCKET HEAD CAP SCREW:24
- Mate:287: L gusset:9 ↔ 1.5in 92196A251_18-8 STAINLESS STEEL SOCKET HEAD CAP SCREW:38
- Mate:288: L gusset:9 ↔ 1.5in 92196A251_18-8 STAINLESS STEEL SOCKET HEAD CAP SCREW:13
- Mate:289: L gusset:8 ↔ 1.5in 92196A251_18-8 STAINLESS STEEL SOCKET HEAD CAP SCREW:43
- Mate:291: L gusset:8 ↔ 1.5in 92196A251_18-8 STAINLESS STEEL SOCKET HEAD CAP SCREW:25
- Mate:292: L gusset:8 ↔ 1.5in 92196A251_18-8 STAINLESS STEEL SOCKET HEAD CAP SCREW:36
- Mate:293: L gusset:8 ↔ 1.5in 92196A251_18-8 STAINLESS STEEL SOCKET HEAD CAP SCREW:35
- Mate:296: L gusset:10 ↔ 1.5in 92196A251_18-8 STAINLESS STEEL SOCKET HEAD CAP SCREW:34
- Mate:297: L gusset:10 ↔ 1.5in 92196A251_18-8 STAINLESS STEEL SOCKET HEAD CAP SCREW:15
- Mate:298: L gusset:10 ↔ 1.5in 92196A251_18-8 STAINLESS STEEL SOCKET HEAD CAP SCREW:17
- Mate:300: 24in Vertical 1x1 Beam:3 ↔ LV Gusset:2
- Mate:301: 25in Horizontal 1x1 Beam:1 ↔ LV Gusset:2
- Mate:302: 25in Horizontal 1x1 Beam:1 ↔ LV Gusset:2
- Mate:303: 25in Horizontal 1x1 Beam:1 ↔ LV Gusset:2
- Mate:304: 24in Vertical 1x1 Beam:3 ↔ LV Gusset:2
- Mate:305: 24in Vertical 1x1 Beam:3 ↔ LV Gusset:2
- Mate:306: 24in Vertical 1x1 Beam:4 ↔ LV Gusset:1
- Mate:307: 25in Horizontal 1x1 Beam:2 ↔ LV Gusset:1
- Mate:308: 25in Horizontal 1x1 Beam:2 ↔ LV Gusset:1
- Mate:309: 25in Horizontal 1x1 Beam:2 ↔ LV Gusset:1
- Mate:310: 24in Vertical 1x1 Beam:4 ↔ LV Gusset:1
- Mate:311: 24in Vertical 1x1 Beam:4 ↔ LV Gusset:1
- Flush:129: 25in Horizontal 1x1 Beam:2 ↔ LV Gusset:1
- Flush:130: 24in Vertical 1x1 Beam:4 ↔ LV Gusset:1
- Flush:131: 24in Vertical 1x1 Beam:4 ↔ LV Gusset:1
- Flush:132: 25in Horizontal 1x1 Beam:2 ↔ LV Gusset:1
- Flush:133: 25in Horizontal 1x1 Beam:1 ↔ LV Gusset:2
- Flush:134: 24in Vertical 1x1 Beam:3 ↔ LV Gusset:2
- Flush:135: 24in Vertical 1x1 Beam:3 ↔ LV Gusset:2
- Flush:136: 25in Horizontal 1x1 Beam:1 ↔ LV Gusset:2
- Mate:312: 1.5in 92196A251_18-8 STAINLESS STEEL SOCKET HEAD CAP SCREW:7 ↔ LV Gusset:2
- Mate:313: 1.5in 92196A251_18-8 STAINLESS STEEL SOCKET HEAD CAP SCREW:11 ↔ LV Gusset:2
- Mate:314: 1.5in 92196A251_18-8 STAINLESS STEEL SOCKET HEAD CAP SCREW:11 ↔ LV Gusset:2
- Mate:315: 1.5in 92196A251_18-8 STAINLESS STEEL SOCKET HEAD CAP SCREW:7 ↔ LV Gusset:2
- Mate:316: 1.5in 92196A251_18-8 STAINLESS STEEL SOCKET HEAD CAP SCREW:14 ↔ LV Gusset:2
- Mate:317: 1.5in 92196A251_18-8 STAINLESS STEEL SOCKET HEAD CAP SCREW:2 ↔ LV Gusset:2
- Mate:318: 1.5in 92196A251_18-8 STAINLESS STEEL SOCKET HEAD CAP SCREW:14 ↔ LV Gusset:2
- Mate:319: 1.5in 92196A251_18-8 STAINLESS STEEL SOCKET HEAD CAP SCREW:2 ↔ LV Gusset:2
- Mate:320: 1.5in 92196A251_18-8 STAINLESS STEEL SOCKET HEAD CAP SCREW:1 ↔ LV Gusset:1
- Mate:321: 1.5in 92196A251_18-8 STAINLESS STEEL SOCKET HEAD CAP SCREW:20 ↔ LV Gusset:1
- Mate:322: 1.5in 92196A251_18-8 STAINLESS STEEL SOCKET HEAD CAP SCREW:1 ↔ LV Gusset:1
- Mate:323: 1.5in 92196A251_18-8 STAINLESS STEEL SOCKET HEAD CAP SCREW:20 ↔ LV Gusset:1
- Mate:324: 1.5in 92196A251_18-8 STAINLESS STEEL SOCKET HEAD CAP SCREW:3 ↔ LV Gusset:1
- Mate:325: 1.5in 92196A251_18-8 STAINLESS STEEL SOCKET HEAD CAP SCREW:8 ↔ LV Gusset:1
- Mate:326: 1.5in 92196A251_18-8 STAINLESS STEEL SOCKET HEAD CAP SCREW:8 ↔ LV Gusset:1
- Mate:327: 1.5in 92196A251_18-8 STAINLESS STEEL SOCKET HEAD CAP SCREW:3 ↔ LV Gusset:1
- Mate:328: L gusset:10 ↔ 1.5in 92196A251_18-8 STAINLESS STEEL SOCKET HEAD CAP SCREW:34
- Mate:329: L gusset:10 ↔ 1.5in 92196A251_18-8 STAINLESS STEEL SOCKET HEAD CAP SCREW:15
- Mate:330: L gusset:10 ↔ 1.5in 92196A251_18-8 STAINLESS STEEL SOCKET HEAD CAP SCREW:17
- Mate:332: L gusset:13 ↔ 1.5in 92196A251_18-8 STAINLESS STEEL SOCKET HEAD CAP SCREW:12
- Mate:333: L gusset:13 ↔ 1.5in 92196A251_18-8 STAINLESS STEEL SOCKET HEAD CAP SCREW:26
- Mate:334: L gusset:13 ↔ 1.5in 92196A251_18-8 STAINLESS STEEL SOCKET HEAD CAP SCREW:22
- Mate:335: L gusset:13 ↔ 1.5in 92196A251_18-8 STAINLESS STEEL SOCKET HEAD CAP SCREW:30
- Mate:336: L gusset:13 ↔ 1.5in 92196A251_18-8 STAINLESS STEEL SOCKET HEAD CAP SCREW:18
- Mate:337: L gusset:10 ↔ 1.5in 92196A251_18-8 STAINLESS STEEL SOCKET HEAD CAP SCREW:28
- Mate:338: L gusset:10 ↔ 1.5in 92196A251_18-8 STAINLESS STEEL SOCKET HEAD CAP SCREW:28
- Mate:339: L gusset:15 ↔ 1.5in 92196A251_18-8 STAINLESS STEEL SOCKET HEAD CAP SCREW:21
- Mate:340: L gusset:15 ↔ 1.5in 92196A251_18-8 STAINLESS STEEL SOCKET HEAD CAP SCREW:21
- Mate:341: L gusset:15 ↔ 1.5in 92196A251_18-8 STAINLESS STEEL SOCKET HEAD CAP SCREW:5
- Mate:342: L gusset:15 ↔ 1.5in 92196A251_18-8 STAINLESS STEEL SOCKET HEAD CAP SCREW:52
- Mate:343: L gusset:19 ↔ 1.5in 92196A251_18-8 STAINLESS STEEL SOCKET HEAD CAP SCREW:51
- Mate:344: L gusset:19 ↔ 1.5in 92196A251_18-8 STAINLESS STEEL SOCKET HEAD CAP SCREW:58
- Mate:345: L gusset:19 ↔ 1.5in 92196A251_18-8 STAINLESS STEEL SOCKET HEAD CAP SCREW:59
- Mate:346: L gusset:19 ↔ 1.5in 92196A251_18-8 STAINLESS STEEL SOCKET HEAD CAP SCREW:59
- Mate:347: L gusset:19 ↔ 1.5in 92196A251_18-8 STAINLESS STEEL SOCKET HEAD CAP SCREW:58
- Mate:348: L gusset:19 ↔ 1.5in 92196A251_18-8 STAINLESS STEEL SOCKET HEAD CAP SCREW:51
- Mate:349: L gusset:15 ↔ 1.5in 92196A251_18-8 STAINLESS STEEL SOCKET HEAD CAP SCREW:52
- Mate:350: L gusset:15 ↔ 1.5in 92196A251_18-8 STAINLESS STEEL SOCKET HEAD CAP SCREW:5
- Mate:351: L gusset:16 ↔ 1.5in 92196A251_18-8 STAINLESS STEEL SOCKET HEAD CAP SCREW:67
- Mate:352: L gusset:16 ↔ 1.5in 92196A251_18-8 STAINLESS STEEL SOCKET HEAD CAP SCREW:61
- Mate:353: L gusset:18 ↔ 1.5in 92196A251_18-8 STAINLESS STEEL SOCKET HEAD CAP SCREW:64
- Mate:354: L gusset:18 ↔ 1.5in 92196A251_18-8 STAINLESS STEEL SOCKET HEAD CAP SCREW:60
- Mate:355: L gusset:18 ↔ 1.5in 92196A251_18-8 STAINLESS STEEL SOCKET HEAD CAP SCREW:60
- Mate:356: L gusset:18 ↔ 1.5in 92196A251_18-8 STAINLESS STEEL SOCKET HEAD CAP SCREW:64
- Mate:357: L gusset:16 ↔ 1.5in 92196A251_18-8 STAINLESS STEEL SOCKET HEAD CAP SCREW:67
- Mate:358: L gusset:16 ↔ 1.5in 92196A251_18-8 STAINLESS STEEL SOCKET HEAD CAP SCREW:61
- Mate:359: L gusset:13 ↔ 1.5in 92196A251_18-8 STAINLESS STEEL SOCKET HEAD CAP SCREW:22
- Mate:360: L gusset:13 ↔ 1.5in 92196A251_18-8 STAINLESS STEEL SOCKET HEAD CAP SCREW:26
- Mate:361: L gusset:13 ↔ 1.5in 92196A251_18-8 STAINLESS STEEL SOCKET HEAD CAP SCREW:12
- Mate:362: L gusset:13 ↔ 1.5in 92196A251_18-8 STAINLESS STEEL SOCKET HEAD CAP SCREW:30
- Mate:363: L gusset:13 ↔ 1.5in 92196A251_18-8 STAINLESS STEEL SOCKET HEAD CAP SCREW:18
- Mate:364: L gusset:11 ↔ 1.5in 92196A251_18-8 STAINLESS STEEL SOCKET HEAD CAP SCREW:6
- Mate:365: L gusset:11 ↔ 1.5in 92196A251_18-8 STAINLESS STEEL SOCKET HEAD CAP SCREW:27
- Mate:366: L gusset:11 ↔ 1.5in 92196A251_18-8 STAINLESS STEEL SOCKET HEAD CAP SCREW:19
- Mate:368: L gusset:11 ↔ 1.5in 92196A251_18-8 STAINLESS STEEL SOCKET HEAD CAP SCREW:31
- Mate:369: L gusset:11 ↔ 1.5in 92196A251_18-8 STAINLESS STEEL SOCKET HEAD CAP SCREW:6
- Mate:370: L gusset:11 ↔ 1.5in 92196A251_18-8 STAINLESS STEEL SOCKET HEAD CAP SCREW:27
- Mate:372: L gusset:11 ↔ 1.5in 92196A251_18-8 STAINLESS STEEL SOCKET HEAD CAP SCREW:19
- Mate:373: L gusset:11 ↔ 1.5in 92196A251_18-8 STAINLESS STEEL SOCKET HEAD CAP SCREW:31
- Mate:376: L gusset:17 ↔ .75in 92196A245_18-8 STAINLESS STEEL SOCKET HEAD CAP SCREW:1
- Mate:377: L gusset:17 ↔ .75in 92196A245_18-8 STAINLESS STEEL SOCKET HEAD CAP SCREW:1
- Mate:380: L gusset:11 ↔ 1.5in 92196A251_18-8 STAINLESS STEEL SOCKET HEAD CAP SCREW:68
- Mate:381: L gusset:11 ↔ 1.5in 92196A251_18-8 STAINLESS STEEL SOCKET HEAD CAP SCREW:68
- Mate:382: L gusset:8 ↔ 1.5in 92196A251_18-8 STAINLESS STEEL SOCKET HEAD CAP SCREW:69
- Mate:383: L gusset:8 ↔ 1.5in 92196A251_18-8 STAINLESS STEEL SOCKET HEAD CAP SCREW:69
- Mate:384: L gusset:20 ↔ .75in 92196A245_18-8 STAINLESS STEEL SOCKET HEAD CAP SCREW:34
- Mate:385: L gusset:20 ↔ .75in 92196A245_18-8 STAINLESS STEEL SOCKET HEAD CAP SCREW:34
- Mate:386: L gusset:20 ↔ .75in 92196A245_18-8 STAINLESS STEEL SOCKET HEAD CAP SCREW:14
- Mate:387: L gusset:20 ↔ .75in 92196A245_18-8 STAINLESS STEEL SOCKET HEAD CAP SCREW:15
- Mate:388: L gusset:17 ↔ .75in 92196A245_18-8 STAINLESS STEEL SOCKET HEAD CAP SCREW:17
- Mate:389: L gusset:17 ↔ .75in 92196A245_18-8 STAINLESS STEEL SOCKET HEAD CAP SCREW:58
- Mate:390: L gusset:17 ↔ .75in 92196A245_18-8 STAINLESS STEEL SOCKET HEAD CAP SCREW:17
- Mate:391: L gusset:17 ↔ .75in 92196A245_18-8 STAINLESS STEEL SOCKET HEAD CAP SCREW:58
- Mate:392: L gusset:20 ↔ .75in 92196A245_18-8 STAINLESS STEEL SOCKET HEAD CAP SCREW:14
- Mate:393: L gusset:20 ↔ .75in 92196A245_18-8 STAINLESS STEEL SOCKET HEAD CAP SCREW:15
- Mate:394: L gusset:17 ↔ 1.5in 92196A251_18-8 STAINLESS STEEL SOCKET HEAD CAP SCREW:54
- Mate:395: L gusset:17 ↔ 1.5in 92196A251_18-8 STAINLESS STEEL SOCKET HEAD CAP SCREW:33
- Mate:396: L gusset:20 ↔ 1.5in 92196A251_18-8 STAINLESS STEEL SOCKET HEAD CAP SCREW:56
- Mate:397: L gusset:20 ↔ 1.5in 92196A251_18-8 STAINLESS STEEL SOCKET HEAD CAP SCREW:50
- Mate:398: L gusset:20 ↔ 1.5in 92196A251_18-8 STAINLESS STEEL SOCKET HEAD CAP SCREW:56
- Mate:399: L gusset:20 ↔ 1.5in 92196A251_18-8 STAINLESS STEEL SOCKET HEAD CAP SCREW:50
- Mate:400: L gusset:17 ↔ 1.5in 92196A251_18-8 STAINLESS STEEL SOCKET HEAD CAP SCREW:54
- Mate:401: L gusset:17 ↔ 1.5in 92196A251_18-8 STAINLESS STEEL SOCKET HEAD CAP SCREW:33
